# Autodesk Inventor assembly: 174370 HNC-40_(50)
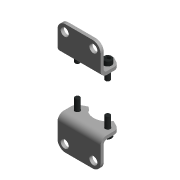
[picture p0: Inventor's stored thumbnail of the model, 180x180]
Saved by Autodesk Inventor 2021 (Build 250183000, 183)
## iProperties
Part Number: 174370 HNC-40_(50)
Catalog Web Link: www.cadenas.de
Description: HNC-Foot mounting
Vendor: FESTO
Document SubType Name: Assembly
Designer: partserver
Manufacturer: FESTO
Mass: 193 g
Surface Area: 157.635 cm^2
Volume: 24.344 cm^3
Density: 7.92804 g/cm^3
Category: PARTsolutions
Company: FESTO
PSOL_IDENT_0: {ATYP=ASSISTANT},{DATA=script=$CADENAS_DATA/23d-libs/festo/webfesto.vbb&M_FAMILY=HNC&M_GROUP=01&M_PA
PSOL_IDENT_1: RTNO=174370&IDCODE1=HNC-40&IDCODE2=&customer_number_cns=&MATES=1&LOD=HI&LOCKERP=0&SINGLEPART=1}
NB: 174370 HNC-40_(50)
NN: HNC
NT: Foot mounting
NBSYN: $TNR. $TYP._($DIST.)
LINA: 174370 HNC-40
CATALOG: Festo
TNR: 174370
TYP: HNC-40
DIST: 50
AB: 10
AH: 36
AW: 37
AT: 4
AU: 28
D2: 6.6
E: 54
LG: 18.5
R1: 17.5
R2: 8
TG: 38
TG2: 19
TR: 36
CNSMASSEXACT: 0.193
SUPPLIER: FESTO
ARTICLENO: 174370 HNC-40_(50)
BOMINFO: 174370 HNC-40
CREATOR: CADENAS GmbH
Title: 174370 HNC-40
Author: Cadenas PARTsolutions
Comments: Foot mounting
## Documents named in this file (3)
- C:\Users\Santiago Suárez\Documents\GitHub\Dis.-Mecatronico-E6\inventor proyecto\ActuadorAvance\AIS2021\174370 HNC-40_(50).iam
- C:\Users\Santiago Suárez\Documents\GitHub\Dis.-Mecatronico-E6\inventor proyecto\ActuadorAvance\AIS2021\174370 HNC-40---(F).ipt
- C:\Users\Santiago Suárez\Documents\GitHub\Dis.-Mecatronico-E6\inventor proyecto\ActuadorAvance\AIS2021\DIN-912 - M6x18(F).ipt
## Components (6 placed, 2 different names)
1. 174370 HNC-40---(F):1 — HNC_1_Z@1 <-> HNC_1_Z@2, HNC_1_YZ@1 <-> HNC_1_YZ@2, HNC_3_XY@1 <-> ANBAU_XY@5, HNC_3_Z@1 <-> ANBAU_Z@5, HNC_2_XY@1 <-> ANBAU_XY@6, HNC_2_Z@1 <-> ANBAU_Z@6, HNC_2_YZ@1 <-> ANBAU_YZ@6
2. 174370 HNC-40---(F):2 — HNC_1_Z@1 <-> HNC_1_Z@2, HNC_1_YZ@1 <-> HNC_1_YZ@2, HNC_3_XY@2 <-> ANBAU_XY@3, HNC_3_Z@2 <-> ANBAU_Z@3, HNC_2_XY@2 <-> ANBAU_XY@4, HNC_2_Z@2 <-> ANBAU_Z@4
3. DIN-912 - M6x18(F):1 — HNC_3_XY@2 <-> ANBAU_XY@3, HNC_3_Z@2 <-> ANBAU_Z@3
4. DIN-912 - M6x18(F):2 — HNC_2_XY@2 <-> ANBAU_XY@4, HNC_2_Z@2 <-> ANBAU_Z@4
5. DIN-912 - M6x18(F):3 — HNC_3_XY@1 <-> ANBAU_XY@5, HNC_3_Z@1 <-> ANBAU_Z@5
6. DIN-912 - M6x18(F):4 — HNC_2_XY@1 <-> ANBAU_XY@6, HNC_2_Z@1 <-> ANBAU_Z@6, HNC_2_YZ@1 <-> ANBAU_YZ@6
## Relationships (11: Mate 5, Flush 4, Angle 2)
- HNC_1_Z@1 <-> HNC_1_Z@2 [Mate]: 174370 HNC-40---(F):1 ↔ 174370 HNC-40---(F):2
- HNC_1_YZ@1 <-> HNC_1_YZ@2 [Angle] (180 deg): 174370 HNC-40---(F):1 ↔ 174370 HNC-40---(F):2
- HNC_3_XY@2 <-> ANBAU_XY@3 [Flush]: 174370 HNC-40---(F):2 ↔ DIN-912 - M6x18(F):1
- HNC_3_Z@2 <-> ANBAU_Z@3 [Mate]: 174370 HNC-40---(F):2 ↔ DIN-912 - M6x18(F):1
- HNC_2_XY@2 <-> ANBAU_XY@4 [Flush]: 174370 HNC-40---(F):2 ↔ DIN-912 - M6x18(F):2
- HNC_2_Z@2 <-> ANBAU_Z@4 [Mate]: 174370 HNC-40---(F):2 ↔ DIN-912 - M6x18(F):2
- HNC_3_XY@1 <-> ANBAU_XY@5 [Flush]: 174370 HNC-40---(F):1 ↔ DIN-912 - M6x18(F):3
- HNC_3_Z@1 <-> ANBAU_Z@5 [Mate]: 174370 HNC-40---(F):1 ↔ DIN-912 - M6x18(F):3
- HNC_2_XY@1 <-> ANBAU_XY@6 [Flush]: 174370 HNC-40---(F):1 ↔ DIN-912 - M6x18(F):4
- HNC_2_Z@1 <-> ANBAU_Z@6 [Mate]: 174370 HNC-40---(F):1 ↔ DIN-912 - M6x18(F):4
- HNC_2_YZ@1 <-> ANBAU_YZ@6 [Angle] (0 deg): 174370 HNC-40---(F):1 ↔ DIN-912 - M6x18(F):4
